# Autodesk Inventor assembly: MP1
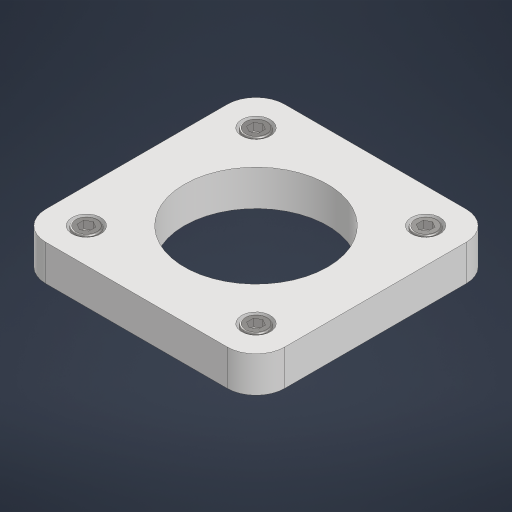
[picture p0: Inventor's stored thumbnail of the model, 512x512]
Saved by Autodesk Inventor 2024.1 (Build 281209000, 209)
## iProperties
Created: 2024-02-20
Part Number: MP1
Document SubType Name: Assembly
Designer: fablabadmin
Author: fablabadmin
## Documents named in this file (3)
- C:\Users\fablabadmin\Documents\_Benjamin_S\_3dCAD\HHVerkstad\MountPlate\MP1.iam
- C:\Users\fablabadmin\Documents\_Benjamin_S\_3dCAD\HHVerkstad\MountPlate\MP1-1001.ipt
- C:\Users\fablabadmin\Documents\Inventor\Content Center Files\R2024\en-US\AS 1420\AS 1420 - 1973 - M6 x 16.ipt
## Components (5 placed, 2 different names)
1. MP1-1001:1 — Insert:1, Insert:2, Insert:3, Insert:4
2. AS 1420 - Metric M6 x 16:1 — Insert:1
3. AS 1420 - Metric M6 x 16:2 — Insert:2
4. AS 1420 - Metric M6 x 16:3 — Insert:3
5. AS 1420 - Metric M6 x 16:4 — Insert:4
## Relationships (4: Insert 4)
- Insert:1: MP1-1001:1 ↔ AS 1420 - Metric M6 x 16:1
- Insert:2: MP1-1001:1 ↔ AS 1420 - Metric M6 x 16:2
- Insert:3: MP1-1001:1 ↔ AS 1420 - Metric M6 x 16:3
- Insert:4: MP1-1001:1 ↔ AS 1420 - Metric M6 x 16:4
